# Autodesk Inventor assembly: Floor_System
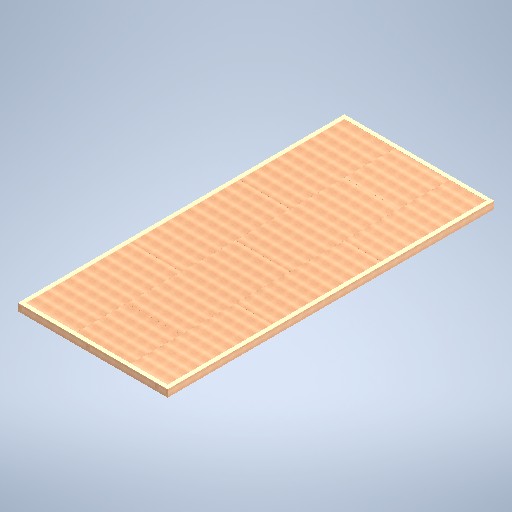
[picture p0: Inventor's stored thumbnail of the model, 512x512]
Saved by Autodesk Inventor 2025 (Build 290162010, 162A)
## iProperties
Created: 2024-10-12
Part Number: Floor_System
Document SubType Name: Assembly
Designer: Tom
Author: Tom
## Documents named in this file (8)
- C:\Users\Tom\Documents\Inventor\Mobility\Additional_Building\Floor_System.iam
- C:\Users\Tom\Documents\Inventor\Mobility\Additional_Building\Beam.ipt
- C:\Users\Tom\Documents\Inventor\Mobility\Additional_Building\Joist_With_Length_56.75_Inches.ipt
- C:\Users\Tom\Documents\Inventor\Mobility\Additional_Building\Joist_With_Length_6.5_Inches.ipt
- C:\Users\Tom\Documents\Inventor\Mobility\Additional_Building\Joist_With_Length_144_Inches.ipt
- C:\Users\Tom\Documents\Inventor\Mobility\Additional_Building\Subfloor.iam
- C:\Users\Tom\Documents\Inventor\Mobility\Additional_Building\Sill_Seal_With_Length_288_Inches.ipt
- C:\Users\Tom\Documents\Inventor\Mobility\Additional_Building\Sill_Seal_With_Length_125_Inches.ipt
## Components (70 placed, 7 different names)
1. Subfloor:1 [sub-assembly] — Mate:6, Flush:11, Flush:12, Mate:7, Flush:13, Flush:14, Mate:8, Flush:15
2. Beam:1
3. Beam:2 — Mate:1, Flush:1, Flush:2, Mate:6, Flush:12, Mate:10, Flush:16
4. Beam:3
5. Beam:4
6. Beam:5
7. Beam:6 — Mate:3, Flush:5, Flush:6, Flush:11, Mate:12, Flush:17
8. Joist_With_Length_144_Inches:1 — Mate:5, Flush:9, Flush:10
9. Joist_With_Length_144_Inches:2
10. Sill_Seal_With_Length_288_Inches:1 — Mate:7, Flush:13, Flush:14, Mate:9
11. Sill_Seal_With_Length_288_Inches:2
12. Sill_Seal_With_Length_125_Inches:1 — Mate:8, Mate:9, Flush:15
13. Sill_Seal_With_Length_125_Inches:2
14. Joist_With_Length_56.75_Inches:2 — Mate:10, Flush:16, Flush:18
15. Joist_With_Length_56.75_Inches:4
16. Joist_With_Length_56.75_Inches:5
17. Joist_With_Length_56.75_Inches:6
18. Joist_With_Length_56.75_Inches:7
19. Joist_With_Length_56.75_Inches:8
20. Joist_With_Length_56.75_Inches:9
21. Joist_With_Length_56.75_Inches:10
22. Joist_With_Length_56.75_Inches:11
23. Joist_With_Length_56.75_Inches:12
24. Joist_With_Length_56.75_Inches:13
25. Joist_With_Length_56.75_Inches:14
26. Joist_With_Length_56.75_Inches:15
27. Joist_With_Length_56.75_Inches:16
28. Joist_With_Length_56.75_Inches:17
29. Joist_With_Length_56.75_Inches:18
30. Joist_With_Length_56.75_Inches:19
31. Joist_With_Length_56.75_Inches:23
32. Joist_With_Length_56.75_Inches:24
33. Joist_With_Length_56.75_Inches:25
34. Joist_With_Length_56.75_Inches:26
35. Joist_With_Length_56.75_Inches:27
36. Joist_With_Length_56.75_Inches:28
37. Joist_With_Length_56.75_Inches:29
38. Joist_With_Length_56.75_Inches:30
39. Joist_With_Length_56.75_Inches:31
40. Joist_With_Length_56.75_Inches:32
41. Joist_With_Length_56.75_Inches:33
42. Joist_With_Length_56.75_Inches:34
43. Joist_With_Length_56.75_Inches:35
44. Joist_With_Length_56.75_Inches:36
45. Joist_With_Length_56.75_Inches:37
46. Joist_With_Length_56.75_Inches:38
47. Joist_With_Length_56.75_Inches:39
48. Joist_With_Length_6.5_Inches:1 — Mate:3, Flush:5, Flush:6, Mate:5, Flush:9, Flush:10, Flush:19
49. Joist_With_Length_6.5_Inches:2
50. Joist_With_Length_6.5_Inches:3 — Mate:12, Flush:17, Flush:19
51. Joist_With_Length_6.5_Inches:4
52. Joist_With_Length_6.5_Inches:5
53. Joist_With_Length_6.5_Inches:6
54. Joist_With_Length_6.5_Inches:7
55. Joist_With_Length_6.5_Inches:8
56. Joist_With_Length_6.5_Inches:9
57. Joist_With_Length_6.5_Inches:10
58. Joist_With_Length_6.5_Inches:11
59. Joist_With_Length_6.5_Inches:12
60. Joist_With_Length_6.5_Inches:13
61. Joist_With_Length_6.5_Inches:14
62. Joist_With_Length_6.5_Inches:15
63. Joist_With_Length_6.5_Inches:16
64. Joist_With_Length_6.5_Inches:17
65. Joist_With_Length_6.5_Inches:18
66. Joist_With_Length_6.5_Inches:19
67. Joist_With_Length_56.75_Inches:1 — Mate:1, Flush:1, Flush:2, Flush:18
68. Joist_With_Length_56.75_Inches:3
69. Joist_With_Length_56.75_Inches:21
70. Joist_With_Length_56.75_Inches:22
## Component patterns: (6 elements, first: Beam:1), (2 elements, first: Joist_With_Length_144_Inches:1), (2 elements, first: Sill_Seal_With_Length_288_Inches:1), (2 elements, first: Sill_Seal_With_Length_125_Inches:1), (34 elements, first: Joist_With_Length_56.75_Inches:2), (2 elements), (2 elements, first: Joist_With_Length_6.5_Inches:1), (17 elements, first: Joist_With_Length_6.5_Inches:3), (2 elements, first: Joist_With_Length_56.75_Inches:1), Component Pattern 8:2 (2 elements)
## Relationships (24: Flush 15, Mate 9)
- Mate:1: Beam:2 ↔ Joist_With_Length_56.75_Inches:1
- Flush:1: Beam:2 ↔ Joist_With_Length_56.75_Inches:1
- Flush:2: Beam:2 ↔ Joist_With_Length_56.75_Inches:1
- Mate:3: Beam:6 ↔ Joist_With_Length_6.5_Inches:1
- Flush:5: Beam:6 ↔ Joist_With_Length_6.5_Inches:1
- Flush:6: Beam:6 ↔ Joist_With_Length_6.5_Inches:1
- Mate:5: Joist_With_Length_144_Inches:1 ↔ Joist_With_Length_6.5_Inches:1
- Flush:9: Joist_With_Length_144_Inches:1 ↔ Joist_With_Length_6.5_Inches:1
- Flush:10: Joist_With_Length_144_Inches:1 ↔ Joist_With_Length_6.5_Inches:1
- Mate:6: Subfloor:1 ↔ Beam:2
- Flush:11: Subfloor:1 ↔ Beam:6
- Flush:12: Subfloor:1 ↔ Beam:2
- Mate:7: Subfloor:1 ↔ Sill_Seal_With_Length_288_Inches:1
- Flush:13: Subfloor:1 ↔ Sill_Seal_With_Length_288_Inches:1
- Flush:14: Subfloor:1 ↔ Sill_Seal_With_Length_288_Inches:1
- Mate:8: Subfloor:1 ↔ Sill_Seal_With_Length_125_Inches:1
- Mate:9: Sill_Seal_With_Length_288_Inches:1 ↔ Sill_Seal_With_Length_125_Inches:1
- Flush:15: Subfloor:1 ↔ Sill_Seal_With_Length_125_Inches:1
- Mate:10: Beam:2 ↔ Joist_With_Length_56.75_Inches:2
- Flush:16: Beam:2 ↔ Joist_With_Length_56.75_Inches:2
- Mate:12: Beam:6 ↔ Joist_With_Length_6.5_Inches:3
- Flush:17: Beam:6 ↔ Joist_With_Length_6.5_Inches:3
- Flush:18 (387.35 mm): Joist_With_Length_56.75_Inches:2 ↔ Joist_With_Length_56.75_Inches:1
- Flush:19 (387.35 mm): Joist_With_Length_6.5_Inches:1 ↔ Joist_With_Length_6.5_Inches:3
